# Autodesk Inventor assembly: Limit switch top + mount left
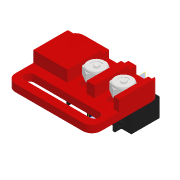
[picture p0: Inventor's stored thumbnail of the model, 180x180]
Saved by Autodesk Inventor 2020 (Build 240168000, 168)
## iProperties
Created: 2019-11-30
Part Number: Limit switch top + mount left
Document SubType Name: Assembly
Designer: ball
Author: ball
## Documents named in this file (5)
- C:\FTC\FTC8863CAD\2019 Robot\Delivery\Limit switch top + mount left.iam
- C:\FTC\FTC8863CAD\2019 Robot\Delivery\Limit switch mount top nut well.ipt
- C:\FTC\FTC8863CAD\Actobotics\605 parts\605630.ipt
- C:\FTC\FTC8863CAD\StepLibraries\Screws\2-56 x .5 TRUSS HEAD PHILLIPS MACHINE SCREW.ipt
- C:\FTC\FTC8863CAD\StepLibraries\Nuts\2-56 NYLON-INSERT LOCKNUT.ipt
## Components (6 placed, 4 different names)
1. Limit switch mount top nut well:1 — Mate:1, Mate:2, Mate:3, Flush:1, Mate:8, Angle:1, Mate:10, Angle:2
2. 605630:1 — Mate:1, Mate:2, Mate:3, Flush:1, Mate:4, Mate:5, Mate:6, Mate:7
3. 2-56 x .5 TRUSS HEAD PHILLIPS MACHINE SCREW:1 — Mate:4, Mate:5, Mate:11
4. 2-56 x .5 TRUSS HEAD PHILLIPS MACHINE SCREW:2 — Mate:6, Mate:7, Mate:9
5. 2-56 NYLON-INSERT LOCKNUT:1 — Mate:8, Mate:9, Angle:1
6. 2-56 NYLON-INSERT LOCKNUT:2 — Mate:10, Mate:11, Angle:2
## Relationships (14: Mate 11, Angle 2, Flush 1)
- Mate:1: Limit switch mount top nut well:1 ↔ 605630:1
- Mate:2: Limit switch mount top nut well:1 ↔ 605630:1
- Mate:3: Limit switch mount top nut well:1 ↔ 605630:1
- Flush:1: Limit switch mount top nut well:1 ↔ 605630:1
- Mate:4: 605630:1 ↔ 2-56 x .5 TRUSS HEAD PHILLIPS MACHINE SCREW:1
- Mate:5: 605630:1 ↔ 2-56 x .5 TRUSS HEAD PHILLIPS MACHINE SCREW:1
- Mate:6: 605630:1 ↔ 2-56 x .5 TRUSS HEAD PHILLIPS MACHINE SCREW:2
- Mate:7: 605630:1 ↔ 2-56 x .5 TRUSS HEAD PHILLIPS MACHINE SCREW:2
- Mate:8: Limit switch mount top nut well:1 ↔ 2-56 NYLON-INSERT LOCKNUT:1
- Mate:9: 2-56 x .5 TRUSS HEAD PHILLIPS MACHINE SCREW:2 ↔ 2-56 NYLON-INSERT LOCKNUT:1
- Angle:1 (0 deg): Limit switch mount top nut well:1 ↔ 2-56 NYLON-INSERT LOCKNUT:1
- Mate:10: Limit switch mount top nut well:1 ↔ 2-56 NYLON-INSERT LOCKNUT:2
- Mate:11: 2-56 x .5 TRUSS HEAD PHILLIPS MACHINE SCREW:1 ↔ 2-56 NYLON-INSERT LOCKNUT:2
- Angle:2 (0 deg): Limit switch mount top nut well:1 ↔ 2-56 NYLON-INSERT LOCKNUT:2
